# Autodesk Inventor assembly: V-Belt transmission
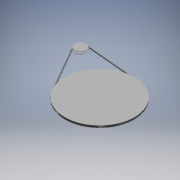
[picture p0: Inventor's stored thumbnail of the model, 180x180]
Saved by Autodesk Inventor 2019 (Build 230136000, 136)
## iProperties
ClientObjectVersion: 1
Created: 2020-02-18
Part Number: V-Belt transmission
Document SubType Name: Assembly
Designer: admin
Author: admin
## Documents named in this file (4)
- C:\Users\admin\Desktop\Exploration\finally_we_are_done_with_stand\Design Accelerator\V-Belt transmission1.iam
- C:\Users\admin\Desktop\Exploration\finally_we_are_done_with_stand\Design Accelerator\V-Belt1.ipt
- C:\Users\admin\Desktop\Exploration\finally_we_are_done_with_stand\Design Accelerator\Grooved Pulley11.ipt
- C:\Users\admin\Desktop\Exploration\finally_we_are_done_with_stand\Design Accelerator\Grooved Pulley21.ipt
## Components (3 placed, 3 different names)
1. Grooved Pulley1:1 — Flush:1, Mate:1, Rotation:1
2. Grooved Pulley2:1 — Flush:2, Mate:2, Rotation:1
3. V-Belt:1 — Flush:1, Mate:1, Flush:2, Mate:2
## Component patterns: (1 elements, first: V-Belt:1)
## Relationships (5: Flush 2, Mate 2, RelateRotation 1)
- Flush:1: Grooved Pulley1:1 ↔ V-Belt:1
- Mate:1: Grooved Pulley1:1 ↔ V-Belt:1
- Flush:2: Grooved Pulley2:1 ↔ V-Belt:1
- Mate:2: Grooved Pulley2:1 ↔ V-Belt:1
- Rotation:1 [RelateRotation] (6.25 ul): Grooved Pulley1:1 ↔ Grooved Pulley2:1
